# Autodesk Inventor assembly: Assembly4 (Piston Sub Assembly)
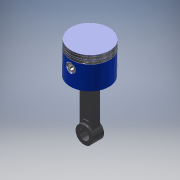
[picture p0: Inventor's stored thumbnail of the model, 180x180]
Saved by Autodesk Inventor 2018 (Build 220112000, 112)
## iProperties
Created: 2023-04-18
Part Number: Assembly4 (Piston Sub Assembly)
Document SubType Name: Assembly
Designer: Habib Mohamed
Author: Habib Mohamed
## Documents named in this file (6)
- D:\Inventor\My projects\Rotary Engine\Assembly\Assembly4 (Piston Sub Assembly).iam
- D:\Inventor\My projects\Rotary Engine\Component 12 (Piston Axis).ipt
- D:\Inventor\My projects\Rotary Engine\Component 6 (Connecting Rod).ipt
- D:\Inventor\My projects\Rotary Engine\Component 8(Piston Ring).ipt
- D:\Inventor\My projects\Rotary Engine\Component 11 (Piston).ipt
- C:\Users\Habib Mohamed\Documents\Inventor\Content Center Files\R2018\en-US\DIN EN ISO 4029\DIN EN ISO 4029 - M2.5  x  2.5.ipt
## Components (7 placed, 5 different names)
1. Component 12 (Piston Axis):1 — Mate:4, Mate:8
2. Component 6 (Connecting Rod):1 — Mate:3, Mate:4, Mate:7
3. Component 8(Piston Ring):1 — Mate:1, Mate:6
4. Component 8(Piston Ring):2 — Mate:2, Mate:5
5. Component 11 (Piston):1 — Mate:1, Mate:2, Mate:3, Mate:5, Mate:6, Mate:7, Mate:8, Mate:9, Mate:10, Flush:1, Flush:2
6. DIN EN ISO 4029 M2.5  x  2.5:1 — Mate:9, Flush:1
7. DIN EN ISO 4029 M2.5  x  2.5:2 — Mate:10, Flush:2
## Relationships (12: Mate 10, Flush 2)
- Mate:1: Component 8(Piston Ring):1 ↔ Component 11 (Piston):1
- Mate:2: Component 8(Piston Ring):2 ↔ Component 11 (Piston):1
- Mate:3: Component 6 (Connecting Rod):1 ↔ Component 11 (Piston):1
- Mate:4: Component 12 (Piston Axis):1 ↔ Component 6 (Connecting Rod):1
- Mate:5: Component 8(Piston Ring):2 ↔ Component 11 (Piston):1
- Mate:6: Component 8(Piston Ring):1 ↔ Component 11 (Piston):1
- Mate:7: Component 6 (Connecting Rod):1 ↔ Component 11 (Piston):1
- Mate:8: Component 12 (Piston Axis):1 ↔ Component 11 (Piston):1
- Mate:9: Component 11 (Piston):1 ↔ DIN EN ISO 4029 M2.5  x  2.5:1
- Mate:10: Component 11 (Piston):1 ↔ DIN EN ISO 4029 M2.5  x  2.5:2
- Flush:1: Component 11 (Piston):1 ↔ DIN EN ISO 4029 M2.5  x  2.5:1
- Flush:2: Component 11 (Piston):1 ↔ DIN EN ISO 4029 M2.5  x  2.5:2
